# Autodesk Inventor assembly: mobile_robot
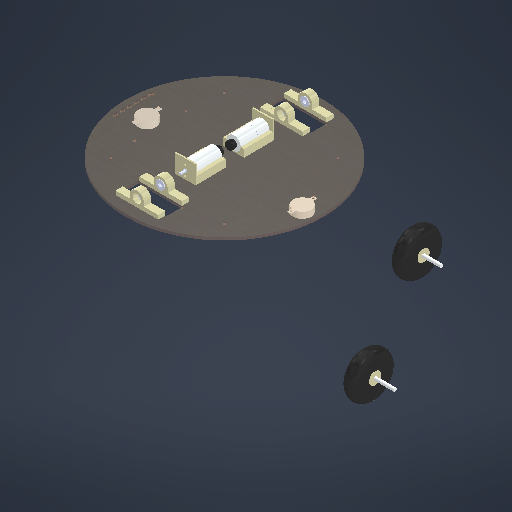
[picture p0: Inventor's stored thumbnail of the model, 512x512]
Saved by Autodesk Inventor 2026 (Build 300175050, 175E)
## iProperties
Created: 2025-06-04
Part Number: mobile_robot
Document SubType Name: Assembly
Designer: satom
Author: satom
## Documents named in this file (10)
- C:\Users\satom\Desktop\Robot\CAD\Inventor\mobile_robot.iam
- C:\Users\satom\Desktop\Robot\CAD\Inventor\C - Chassis\layer1.ipt
- C:\Users\satom\Desktop\Robot\CAD\Inventor\D - DriveTrain\wheel_bearing.ipt
- C:\Users\satom\Desktop\Robot\CAD\Inventor\D - DriveTrain\wheel_mount.ipt
- C:\Users\satom\Desktop\Robot\CAD\Inventor\D - DriveTrain\motor_holder.ipt
- C:\Users\satom\Desktop\Robot\CAD\Inventor\solidworks\D - DriveTrain\ball_caster\ball_caster\ball_caster.ipt
- C:\Users\satom\Desktop\Robot\CAD\Inventor\solidworks\D - DriveTrain\motor\motor\motor.ipt
- C:\Users\satom\Desktop\Robot\CAD\Inventor\solidworks\D - DriveTrain\wheel\wheel\wheel.ipt
- C:\Users\satom\Desktop\Robot\CAD\Inventor\solidworks\D - DriveTrain\drive_shaft\drive_shaft\drive_shaft.ipt
- C:\Users\satom\Desktop\Robot\CAD\Inventor\solidworks\D - DriveTrain\ball_bearing\ball_bearing\ball_bearing.ipt
## Components (23 placed, 9 different names)
1. layer1:1 — Mate:1, Mate:2, Mate:3, Mate:4, Mate:5, Mate:6, Mate:7, Mate:8, Mate:9, Mate:10, Mate:11, Mate:12, Mate:13, Mate:14, Mate:15, Mate:16, Mate:17, Mate:18, Mate:19, Mate:20, Mate:21, Mate:22, Mate:23
2. wheel_bearing:1 — Mate:7, Mate:8, Mate:16, Mate:40, Mate:41
3. wheel_mount:1 — Mate:32, Mate:33, Flush:2
4. motor_holder:1 — Mate:2, Mate:3, Mate:26, Mate:27
5. wheel_bearing:2 — Mate:9, Mate:10, Mate:14, Mate:15, Mate:46, Mate:47
6. wheel_mount:2 — Mate:28, Mate:29, Flush:1, Mate:36, Mate:37
7. motor_holder:2 — Mate:1, Mate:4, Mate:24, Mate:25
8. wheel_bearing:3 — Mate:11, Mate:12, Mate:13, Mate:44, Mate:45
9. wheel_mount:3 — Mate:30, Mate:31, Flush:1
10. wheel_bearing:4 — Mate:5, Mate:6, Mate:17, Mate:42, Mate:43
11. wheel_mount:4 — Mate:34, Mate:35, Flush:2, Mate:38, Mate:39
12. ball_caster:1 — Mate:19, Mate:22, Mate:23
13. ball_caster:2 — Mate:18, Mate:20, Mate:21
14. motor:1 — Mate:24, Mate:25
15. motor:2 — Mate:26, Mate:27
16. wheel:1 — Mate:32, Mate:33, Mate:34, Mate:35
17. wheel:2 — Mate:28, Mate:29, Mate:30, Mate:31
18. drive_shaft:1 — Mate:38, Mate:39
19. drive_shaft:2 — Mate:36, Mate:37
20. ball_bearing:1 — Mate:42, Mate:43
21. ball_bearing:2 — Mate:40, Mate:41
22. ball_bearing:3 — Mate:44, Mate:45
23. ball_bearing:4 — Mate:46, Mate:47
## Relationships (49: Mate 47, Flush 2)
- Mate:1: layer1:1 ↔ motor_holder:2
- Mate:2: layer1:1 ↔ motor_holder:1
- Mate:3: layer1:1 ↔ motor_holder:1
- Mate:4: layer1:1 ↔ motor_holder:2
- Mate:5: layer1:1 ↔ wheel_bearing:4
- Mate:6: layer1:1 ↔ wheel_bearing:4
- Mate:7: layer1:1 ↔ wheel_bearing:1
- Mate:8: layer1:1 ↔ wheel_bearing:1
- Mate:9: layer1:1 ↔ wheel_bearing:2
- Mate:10: layer1:1 ↔ wheel_bearing:2
- Mate:11: layer1:1 ↔ wheel_bearing:3
- Mate:12: layer1:1 ↔ wheel_bearing:3
- Mate:13: layer1:1 ↔ wheel_bearing:3
- Mate:14: layer1:1 ↔ wheel_bearing:2
- Mate:15: layer1:1 ↔ wheel_bearing:2
- Mate:16: layer1:1 ↔ wheel_bearing:1
- Mate:17: layer1:1 ↔ wheel_bearing:4
- Mate:18: layer1:1 ↔ ball_caster:2
- Mate:19: layer1:1 ↔ ball_caster:1
- Mate:20: layer1:1 ↔ ball_caster:2
- Mate:21: layer1:1 ↔ ball_caster:2
- Mate:22: layer1:1 ↔ ball_caster:1
- Mate:23: layer1:1 ↔ ball_caster:1
- Mate:24: motor_holder:2 ↔ motor:1
- Mate:25: motor_holder:2 ↔ motor:1
- Mate:26: motor_holder:1 ↔ motor:2
- Mate:27: motor_holder:1 ↔ motor:2
- Mate:28: wheel_mount:2 ↔ wheel:2
- Mate:29: wheel_mount:2 ↔ wheel:2
- Mate:30: wheel_mount:3 ↔ wheel:2
- Mate:31: wheel_mount:3 ↔ wheel:2
- Flush:1: wheel_mount:2 ↔ wheel_mount:3
- Mate:32: wheel_mount:1 ↔ wheel:1
- Mate:33: wheel_mount:1 ↔ wheel:1
- Mate:34: wheel_mount:4 ↔ wheel:1
- Mate:35: wheel_mount:4 ↔ wheel:1
- Flush:2: wheel_mount:1 ↔ wheel_mount:4
- Mate:36: wheel_mount:2 ↔ drive_shaft:2
- Mate:37: wheel_mount:2 ↔ drive_shaft:2
- Mate:38: wheel_mount:4 ↔ drive_shaft:1
- Mate:39: wheel_mount:4 ↔ drive_shaft:1
- Mate:40: wheel_bearing:1 ↔ ball_bearing:2
- Mate:41: wheel_bearing:1 ↔ ball_bearing:2
- Mate:42: wheel_bearing:4 ↔ ball_bearing:1
- Mate:43: wheel_bearing:4 ↔ ball_bearing:1
- Mate:44: wheel_bearing:3 ↔ ball_bearing:3
- Mate:45: wheel_bearing:3 ↔ ball_bearing:3
- Mate:46: wheel_bearing:2 ↔ ball_bearing:4
- Mate:47: wheel_bearing:2 ↔ ball_bearing:4
